# Autodesk Inventor assembly: axis5_6 v2
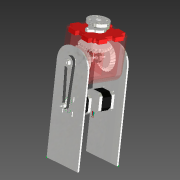
[picture p0: Inventor's stored thumbnail of the model, 180x180]
Saved by Autodesk Inventor 2020 (Build 240168000, 168)
## iProperties
Created: 2020-05-15
Part Number: axis5_6 v2
Document SubType Name: Assembly
Designer: stefa
Author: stefa
## Documents named in this file (8)
- D:\github_gedeeld\BeerMinder\3D-model\axis5_6\axis5_6 v2.iam
- D:\github_gedeeld\BeerMinder\3D-model\pulleys\tandriem32Tnaar16T_lengte240.ipt
- D:\github_gedeeld\BeerMinder\3D-model\pulleys\GT2 Timing Pulley 36T - 8mm as.ipt
- D:\github_gedeeld\BeerMinder\3D-model\stepper motors\42BYG Stepper Motor.ipt
- D:\github_gedeeld\BeerMinder\3D-model\pulleys\GT2 Pulley 16T - 5mm as.ipt
- D:\github_gedeeld\BeerMinder\3D-model\axis5_6\bovenarm - links.ipt
- D:\github_gedeeld\BeerMinder\3D-model\axis5_6\differential gearbox.iam
- D:\github_gedeeld\BeerMinder\3D-model\bearings\lager 8mm - buiten 14 (sven 2 stuks).ipt
## Components (13 placed, 7 different names)
1. tandriem32Tnaar16T_lengte240:1 — Mate:57, Mate:58, Mate:106, Mate:107
2. tandriem32Tnaar16T_lengte240:2 — Mate:60, Mate:89, Mate:94, Mate:100
3. 42BYG Stepper Motor:2 — Mate:96, Mate:108, Flush:12
4. bovenarm - links:1 — Angle:3, Flush:6, Flush:7, Mate:96, Flush:12, Mate:109, Mate:113, Flush:14
5. GT2 Timing Pulley 36T - 8mm as:6 — Mate:57, Mate:58, Mate:110, Flush:16
6. GT2 Timing Pulley 36T - 8mm as:7 — Mate:60, Mate:100, Mate:111, Flush:15
7. bovenarm - links:2 — Flush:6, Flush:7, Mate:99, Mate:102, Flush:10, Mate:103, Mate:104, Mate:105, Mate:112, Flush:13
8. GT2 Pulley 16T - 5mm as:2 — Mate:89, Mate:94, Mate:101, Mate:102
9. GT2 Pulley 16T - 5mm as:3 — Mate:106, Mate:107, Mate:108, Mate:109
10. 42BYG Stepper Motor:3 — Mate:99, Mate:101, Flush:10
11. differential gearbox:1 [sub-assembly] — Mate:110, Mate:111, Mate:114, Mate:115, Flush:15, Flush:16
12. lager 8mm - buiten 14 (sven 2 stuks):1 — Mate:112, Flush:13, Mate:114
13. lager 8mm - buiten 14 (sven 2 stuks):2 — Mate:113, Flush:14, Mate:115
## Relationships (32: Mate 23, Flush 8, Angle 1)
- Angle:3 (0 deg): bovenarm - links:1
- Mate:57 (0.5 mm): tandriem32Tnaar16T_lengte240:1 ↔ GT2 Timing Pulley 36T - 8mm as:6
- Mate:58: tandriem32Tnaar16T_lengte240:1 ↔ GT2 Timing Pulley 36T - 8mm as:6
- Mate:60 (0.5 mm): tandriem32Tnaar16T_lengte240:2 ↔ GT2 Timing Pulley 36T - 8mm as:7
- Flush:6: bovenarm - links:1 ↔ bovenarm - links:2
- Flush:7: bovenarm - links:1 ↔ bovenarm - links:2
- Mate:89 (0.5 mm): tandriem32Tnaar16T_lengte240:2 ↔ GT2 Pulley 16T - 5mm as:2
- Mate:94: tandriem32Tnaar16T_lengte240:2 ↔ GT2 Pulley 16T - 5mm as:2
- Mate:96: 42BYG Stepper Motor:2 ↔ bovenarm - links:1
- Mate:99: bovenarm - links:2 ↔ 42BYG Stepper Motor:3
- Mate:100: tandriem32Tnaar16T_lengte240:2 ↔ GT2 Timing Pulley 36T - 8mm as:7
- Mate:101: GT2 Pulley 16T - 5mm as:2 ↔ 42BYG Stepper Motor:3
- Mate:102 (2 mm): bovenarm - links:2 ↔ GT2 Pulley 16T - 5mm as:2
- Flush:10 (-6.55 mm): bovenarm - links:2 ↔ 42BYG Stepper Motor:3
- Mate:103: bovenarm - links:2
- Mate:104: bovenarm - links:2
- Mate:105: bovenarm - links:2
- Mate:106: tandriem32Tnaar16T_lengte240:1 ↔ GT2 Pulley 16T - 5mm as:3
- Mate:107 (0.5 mm): tandriem32Tnaar16T_lengte240:1 ↔ GT2 Pulley 16T - 5mm as:3
- Mate:108: 42BYG Stepper Motor:2 ↔ GT2 Pulley 16T - 5mm as:3
- Flush:12 (6.8 mm): 42BYG Stepper Motor:2 ↔ bovenarm - links:1
- Mate:109 (2 mm): bovenarm - links:1 ↔ GT2 Pulley 16T - 5mm as:3
- Mate:110: GT2 Timing Pulley 36T - 8mm as:6 ↔ differential gearbox:1
- Mate:111: GT2 Timing Pulley 36T - 8mm as:7 ↔ differential gearbox:1
- Mate:112: bovenarm - links:2 ↔ lager 8mm - buiten 14 (sven 2 stuks):1
- Flush:13: bovenarm - links:2 ↔ lager 8mm - buiten 14 (sven 2 stuks):1
- Mate:113: bovenarm - links:1 ↔ lager 8mm - buiten 14 (sven 2 stuks):2
- Flush:14: bovenarm - links:1 ↔ lager 8mm - buiten 14 (sven 2 stuks):2
- Mate:114: differential gearbox:1 ↔ lager 8mm - buiten 14 (sven 2 stuks):1
- Mate:115: differential gearbox:1 ↔ lager 8mm - buiten 14 (sven 2 stuks):2
- Flush:15 (-1 mm): GT2 Timing Pulley 36T - 8mm as:7 ↔ differential gearbox:1
- Flush:16 (-1 mm): GT2 Timing Pulley 36T - 8mm as:6 ↔ differential gearbox:1
